# Autodesk Inventor assembly: mpalanteza_assembly
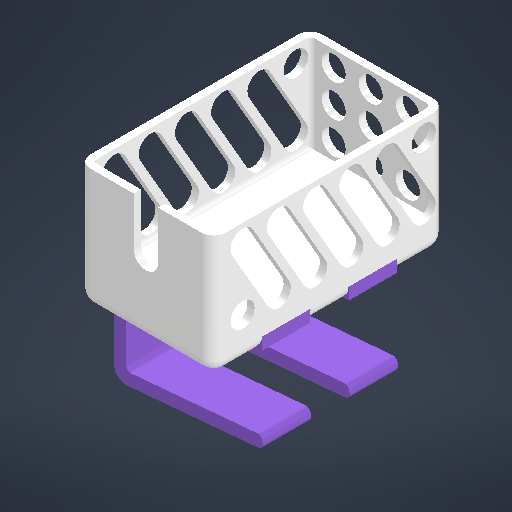
[picture p0: Inventor's stored thumbnail of the model, 512x512]
Saved by Autodesk Inventor 2026.1 (Build 301233020, 233B)
## iProperties
Created: 2026-02-17
Part Number: mpalanteza_assembly
Document SubType Name: Assembly
Designer: ar_mi
Author: ar_mi
## Documents named in this file (3)
- D:\Inventor 2026\mpalanteza_assembly.iam
- D:\Inventor 2026\mpalanteza_clips.ipt
- D:\Inventor 2026\mpalanteza_holder.ipt
## Components (3 placed, 2 different names)
1. mpalanteza_clips:1 — Flush:1, Mate:1, Mate:2
2. mpalanteza_clips:2 — Flush:2, Mate:3, Mate:4
3. mpalanteza_holder:1 — Flush:1, Flush:2, Mate:1, Mate:2, Mate:3, Mate:4
## Relationships (6: Mate 4, Flush 2)
- Flush:1: mpalanteza_clips:1 ↔ mpalanteza_holder:1
- Flush:2: mpalanteza_clips:2 ↔ mpalanteza_holder:1
- Mate:1: mpalanteza_clips:1 ↔ mpalanteza_holder:1
- Mate:2: mpalanteza_clips:1 ↔ mpalanteza_holder:1
- Mate:3: mpalanteza_clips:2 ↔ mpalanteza_holder:1
- Mate:4: mpalanteza_clips:2 ↔ mpalanteza_holder:1
